# Autodesk Inventor assembly: sestaveny dum
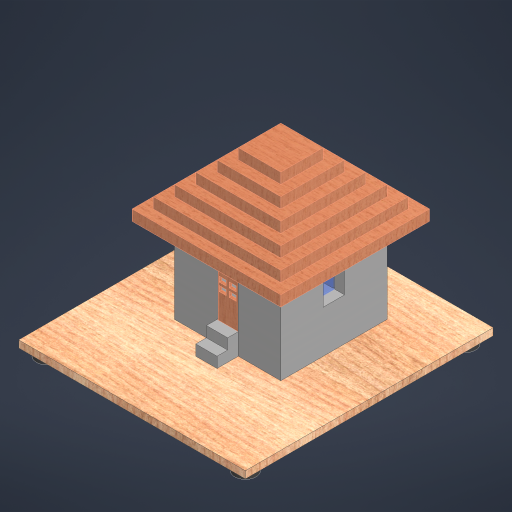
[picture p0: Inventor's stored thumbnail of the model, 512x512]
Saved by Autodesk Inventor 2023 (Build 270158000, 158)
## iProperties
Created: 2022-10-19
Part Number: sestaveny dum
Document SubType Name: Assembly
Designer: zak
Mass: 6542.84 g
Surface Area: 5805.75 cm^2
Volume: 4799.21 cm^3
Density: 1.36331 g/cm^3
Author: zak
## Documents named in this file (7)
- H:\KYB\minecraft baracek\model domu\sestaveny dum.iam
- H:\KYB\minecraft baracek\model domu\deska.ipt
- H:\KYB\minecraft baracek\model domu\steny.ipt
- H:\KYB\minecraft baracek\model domu\strecha.ipt
- H:\KYB\minecraft baracek\model domu\sklo.ipt
- H:\KYB\minecraft baracek\model domu\pacicka.ipt
- H:\KYB\minecraft baracek\model domu\dvere.ipt
## Components (9 placed, 6 different names)
1. deska:1 — Proti sobě:1, Vložit:2, Vložit:3, Proti sobě:9, Vložit:4, Proti sobě:10, Proti sobě:11, Proti sobě:12, Vložit:5, Vložit:6, Vložit:7
2. steny:1 — Proti sobě:1, Proti sobě:3, Proti sobě:4, Proti sobě:5, Vložit:2, Vložit:3, Proti sobě:6, Proti sobě:7, Proti sobě:8, Proti sobě:13, Vložit:8
3. strecha:1 — Proti sobě:3, Proti sobě:4, Proti sobě:5
4. sklo:1 — Proti sobě:6, Proti sobě:7, Proti sobě:8
5. pacicka:1 — Proti sobě:11, Vložit:7
6. pacicka:2 — Proti sobě:12, Vložit:6
7. pacicka:3 — Proti sobě:10, Vložit:5
8. pacicka:4 — Proti sobě:9, Vložit:4
9. dvere:1 — Proti sobě:13, Vložit:8
## Relationships (19: Mate 12, Insert 7)
- Proti sobě:1 [Mate]: deska:1 ↔ steny:1
- Proti sobě:3 [Mate]: steny:1 ↔ strecha:1
- Proti sobě:4 [Mate]: steny:1 ↔ strecha:1
- Proti sobě:5 [Mate]: steny:1 ↔ strecha:1
- Vložit:2 [Insert]: deska:1 ↔ steny:1
- Vložit:3 [Insert]: deska:1 ↔ steny:1
- Proti sobě:6 [Mate]: steny:1 ↔ sklo:1
- Proti sobě:7 [Mate]: steny:1 ↔ sklo:1
- Proti sobě:8 [Mate]: steny:1 ↔ sklo:1
- Proti sobě:9 [Mate]: deska:1 ↔ pacicka:4
- Vložit:4 [Insert]: deska:1 ↔ pacicka:4
- Proti sobě:10 [Mate]: deska:1 ↔ pacicka:3
- Proti sobě:11 [Mate]: deska:1 ↔ pacicka:1
- Proti sobě:12 [Mate]: deska:1 ↔ pacicka:2
- Vložit:5 [Insert]: deska:1 ↔ pacicka:3
- Vložit:6 [Insert]: deska:1 ↔ pacicka:2
- Vložit:7 [Insert]: deska:1 ↔ pacicka:1
- Proti sobě:13 [Mate]: steny:1 ↔ dvere:1
- Vložit:8 [Insert]: steny:1 ↔ dvere:1
